# Autodesk Inventor assembly: Front Lower Arm with pillow ball
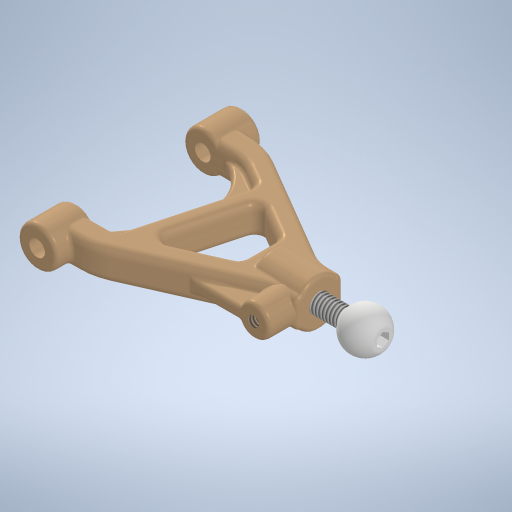
[picture p0: Inventor's stored thumbnail of the model, 512x512]
Saved by Autodesk Inventor 2024 (Build 280153000, 153)
## iProperties
Created: 2023-07-06
Part Number: Front Lower Arm with pillow ball
Document SubType Name: Assembly
Designer: birud
Author: birud
## Documents named in this file (3)
- C:\Users\birud\OneDrive\Desktop\Projects\EG\Front Lower Arm with pillow ball.iam
- C:\Users\birud\OneDrive\Desktop\Projects\EG\Front Lower Arm.ipt
- C:\Users\birud\OneDrive\Desktop\Projects\EG\Pillow Ball.ipt
## Components (2 placed, 2 different names)
1. Front Lower Arm:1 — Mate:1, Mate:2
2. Pillow Ball:1 — Mate:1, Mate:2
## Relationships (2: Mate 2)
- Mate:1: Front Lower Arm:1 ↔ Pillow Ball:1
- Mate:2 (92.075 mm): Front Lower Arm:1 ↔ Pillow Ball:1
